# Autodesk Inventor assembly: Assembly1
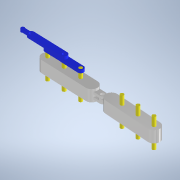
[picture p0: Inventor's stored thumbnail of the model, 180x180]
Saved by Autodesk Inventor 2022 (Build 260153000, 153)
## iProperties
Created: 2022-02-01
Part Number: Assembly1
Document SubType Name: Assembly
Designer: br4ch
Author: br4ch
## Documents named in this file (7)
- C:\Users\br4ch\M-and-Ms\Legs\Assembly1.iam
- C:\Users\br4ch\M-and-Ms\Legs\Part5.ipt
- C:\Users\br4ch\M-and-Ms\Legs\Part6.ipt
- C:\Users\br4ch\M-and-Ms\Legs\Part7.ipt
- C:\Users\br4ch\M-and-Ms\Legs\Part8.ipt
- C:\Users\br4ch\M-and-Ms\Legs\Part9.ipt
- C:\Users\br4ch\M-and-Ms\Legs\Part10.ipt
## Components (12 placed, 6 different names)
1. Part5:1 — Rotational:4, Rotational:11
2. Part6:1 — Rotational:4, Rotational:13
3. Part7:1 — Rotational:10, Rotational:17, Rotational:18, Rotational:19
4. Part8:1 — Rotational:10, Rotational:14, Rotational:15, Rotational:16
5. Part5:2 — Rotational:9, Rotational:12
6. Part9:1 — Rotational:12, Rotational:13
7. Part10:1 — Rotational:14, Rotational:11
8. Part10:2 — Rotational:15
9. Part10:3 — Rotational:16, Rotational:9
10. Part10:4 — Rotational:17
11. Part10:5 — Rotational:19
12. Part10:6 — Rotational:18
## Relationships (12: RevoluteJoint 12)
- Rotational:4 [RevoluteJoint]: Part5:1 ↔ Part6:1
- Rotational:9 [RevoluteJoint]: Part5:2 ↔ Part10:3
- Rotational:10 [RevoluteJoint]: Part7:1 ↔ Part8:1
- Rotational:11 [RevoluteJoint]: Part5:1 ↔ Part10:1
- Rotational:12 [RevoluteJoint]: Part5:2 ↔ Part9:1
- Rotational:13 [RevoluteJoint]: Part6:1 ↔ Part9:1
- Rotational:14 [RevoluteJoint]: Part8:1 ↔ Part10:1
- Rotational:15 [RevoluteJoint]: Part8:1 ↔ Part10:2
- Rotational:16 [RevoluteJoint]: Part8:1 ↔ Part10:3
- Rotational:17 [RevoluteJoint]: Part7:1 ↔ Part10:4
- Rotational:18 [RevoluteJoint]: Part7:1 ↔ Part10:6
- Rotational:19 [RevoluteJoint]: Part7:1 ↔ Part10:5
